# Autodesk Inventor assembly: obudowa_elektroniki_proper
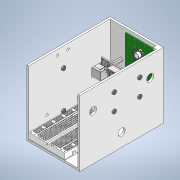
[picture p0: Inventor's stored thumbnail of the model, 180x180]
Saved by Autodesk Inventor 2020 (Build 240168000, 168)
## iProperties
Created: 2020-08-10
Part Number: obudowa_elektroniki_proper
Document SubType Name: Assembly
Designer: Hesekiel
Mass: 257.361 g
Surface Area: 1839.5 cm^2
Volume: 234.13 cm^3
Density: 1.09922 g/cm^3
Author: Hesekiel
## Documents named in this file (12)
- C:\Users\Hesekiel\Desktop\Equatorial-Mount-MUM\Mechanika\Mechanizm elewacji i elektronika Filip\CAD\obudowa_elektroniki_proper.iam
- C:\Users\Hesekiel\Desktop\Equatorial-Mount-MUM\Mechanika\Mechanizm elewacji i elektronika Filip\CAD\Sterownik silnika - Dual TB9051FTG.ipt
- C:\Users\Hesekiel\Desktop\Equatorial-Mount-MUM\Mechanika\Mechanizm elewacji i elektronika Filip\CAD\Konwerter step-down - D24V150FX.ipt
- C:\Users\Hesekiel\Desktop\Equatorial-Mount-MUM\Mechanika\Mechanizm elewacji i elektronika Filip\CAD\obudowa.ipt
- C:\Users\Hesekiel\Desktop\Equatorial-Mount-MUM\Mechanika\Mechanizm elewacji i elektronika Filip\CAD\arduino-uno-r3-1.snapshot.3\arduino uno.iam
- C:\Users\Hesekiel\Desktop\Equatorial-Mount-MUM\Mechanika\Mechanizm elewacji i elektronika Filip\CAD\DIN 912 - M3 x 0.5 x 6 x 4.75.ipt
- C:\Users\Hesekiel\Desktop\Equatorial-Mount-MUM\Mechanika\Mechanizm elewacji i elektronika Filip\CAD\DIN 934 - M3 x 0.5.ipt
- C:\Users\Hesekiel\Desktop\Equatorial-Mount-MUM\Mechanika\Mechanizm elewacji i elektronika Filip\CAD\Standoff_M3_14mm.ipt
- C:\Users\Hesekiel\Desktop\Equatorial-Mount-MUM\Mechanika\Mechanizm elewacji i elektronika Filip\CAD\HalfBreadboard.ipt
- C:\Users\Hesekiel\Desktop\Equatorial-Mount-MUM\Mechanika\Mechanizm elewacji i elektronika Filip\CAD\Battery 18650.ipt
- C:\Users\Hesekiel\Desktop\Equatorial-Mount-MUM\Mechanika\Mechanizm elewacji i elektronika Filip\CAD\battery-holder-for-2x-18650-1.snapshot.2\18650 holder 2x.ipt
- C:\Users\Hesekiel\Desktop\Equatorial-Mount-MUM\Mechanika\Mechanizm elewacji i elektronika Filip\CAD\DIN 912 - M3 x 0.5 x 10 x 8.75.ipt
## Components (39 placed, 11 different names)
1. Sterownik silnika - Dual TB9051FTG:1 — Mate:91, Mate:92, Mate:93, Mate:94, Mate:95, Mate:96, Mate:97
2. Konwerter step-down - D24V150FX:1 — Mate:55, Mate:56, Mate:65, Mate:66, Mate:67, Mate:68, Mate:69, Mate:70, Mate:71, Mate:72, Mate:73
3. obudowa:1 — Mate:1, Mate:2, Mate:30, Mate:31, Mate:32, Mate:33, Mate:34, Mate:35, Mate:36, Mate:37, Mate:39, Mate:40, Mate:41, Mate:42, Mate:44, Mate:50, Mate:51, Mate:52, Mate:55, Mate:56, Mate:57, Mate:58, Mate:59, Mate:60, Mate:61, Mate:62, Mate:63, Mate:64, Mate:75, Mate:76, Mate:77, Mate:81, Mate:85, Mate:86, Mate:88, Mate:91, Mate:92, Mate:95, Mate:99, Mate:100, Flush:3, Mate:101
4. arduino uno:1 [sub-assembly] — Mate:1, Mate:2, Mate:22, Mate:23, Mate:24, Mate:25, Mate:26, Mate:27, Mate:28, Mate:29, Mate:38
5. DIN 912 - replaced by DIN EN ISO 4762 M3 x 6:1 — Mate:22, Mate:23
6. DIN 912 - replaced by DIN EN ISO 4762 M3 x 6:2 — Mate:24, Mate:25
7. DIN 912 - replaced by DIN EN ISO 4762 M3 x 6:3 — Mate:26, Mate:27
8. DIN 912 - replaced by DIN EN ISO 4762 M3 x 6:4 — Mate:28, Mate:29
9. DIN 934 - replaced by DIN EN 24032/28673/28674 M3:1 — Mate:40, Mate:45
10. DIN 934 - replaced by DIN EN 24032/28673/28674 M3:2 — Mate:39, Mate:46
11. DIN 934 - replaced by DIN EN 24032/28673/28674 M3:3 — Mate:41, Mate:44
12. DIN 934 - replaced by DIN EN 24032/28673/28674 M3:4 — Mate:42, Mate:43
13. Standoff_M3_14mm:1 — Mate:30, Mate:31, Mate:38, Mate:43
14. Standoff_M3_14mm:2 — Mate:32, Mate:33
15. Standoff_M3_14mm:3 — Mate:34, Mate:35, Mate:45
16. Standoff_M3_14mm:4 — Mate:36, Mate:37, Mate:46
17. HalfBreadboard:1 — Mate:100, Flush:3, Mate:101
18. Battery 18650:1 — Mate:54, Flush:2
19. Battery 18650:2 — Mate:53, Flush:2
20. 18650 holder 2x:1 — Mate:50, Mate:51, Mate:52, Mate:53, Mate:54, Mate:83, Mate:84, Mate:89
21. DIN 934 - replaced by DIN EN 24032/28673/28674 M3:5 — Mate:57, Mate:61
22. DIN 934 - replaced by DIN EN 24032/28673/28674 M3:6 — Mate:58, Mate:62
23. DIN 934 - replaced by DIN EN 24032/28673/28674 M3:7 — Mate:59, Mate:63, Mate:65
24. DIN 934 - replaced by DIN EN 24032/28673/28674 M3:8 — Mate:60, Mate:64
25. DIN 912 - replaced by DIN EN ISO 4762 M3 x 10:1 — Mate:68, Mate:69, Mate:82
26. DIN 912 - replaced by DIN EN ISO 4762 M3 x 10:2 — Mate:70, Mate:71, Mate:79
27. DIN 912 - replaced by DIN EN ISO 4762 M3 x 10:3 — Mate:72, Mate:73, Mate:78
28. DIN 912 - replaced by DIN EN ISO 4762 M3 x 10:4 — Mate:66, Mate:67, Mate:80
29. DIN 934 - replaced by DIN EN 24032/28673/28674 M3:10 — Mate:75, Mate:79
30. DIN 934 - replaced by DIN EN 24032/28673/28674 M3:11 — Mate:76, Mate:78
31. DIN 934 - replaced by DIN EN 24032/28673/28674 M3:12 — Mate:77, Mate:80
32. DIN 934 - replaced by DIN EN 24032/28673/28674 M3:13 — Mate:81, Mate:82
33. DIN 912 - replaced by DIN EN ISO 4762 M3 x 6:5 — Mate:83, Mate:84, Mate:87
34. DIN 912 - replaced by DIN EN ISO 4762 M3 x 6:6 — Mate:88, Mate:89, Mate:90
35. DIN 934 - replaced by DIN EN 24032/28673/28674 M3:14 — Mate:85, Mate:87
36. DIN 934 - replaced by DIN EN 24032/28673/28674 M3:15 — Mate:86, Mate:90
37. DIN 934 - replaced by DIN EN 24032/28673/28674 M3:16 — Mate:93, Mate:94
38. DIN 912 - replaced by DIN EN ISO 4762 M3 x 10:5 — Mate:96, Mate:97, Mate:98
39. DIN 934 - replaced by DIN EN 24032/28673/28674 M3:17 — Mate:98, Mate:99
## Relationships (80: Mate 78, Flush 2)
- Mate:1: obudowa:1 ↔ arduino uno:1
- Mate:2: obudowa:1 ↔ arduino uno:1
- Mate:22: arduino uno:1 ↔ DIN 912 - replaced by DIN EN ISO 4762 M3 x 6:1
- Mate:23: arduino uno:1 ↔ DIN 912 - replaced by DIN EN ISO 4762 M3 x 6:1
- Mate:24: arduino uno:1 ↔ DIN 912 - replaced by DIN EN ISO 4762 M3 x 6:2
- Mate:25: arduino uno:1 ↔ DIN 912 - replaced by DIN EN ISO 4762 M3 x 6:2
- Mate:26: arduino uno:1 ↔ DIN 912 - replaced by DIN EN ISO 4762 M3 x 6:3
- Mate:27: arduino uno:1 ↔ DIN 912 - replaced by DIN EN ISO 4762 M3 x 6:3
- Mate:28: arduino uno:1 ↔ DIN 912 - replaced by DIN EN ISO 4762 M3 x 6:4
- Mate:29: arduino uno:1 ↔ DIN 912 - replaced by DIN EN ISO 4762 M3 x 6:4
- Mate:30: obudowa:1 ↔ Standoff_M3_14mm:1
- Mate:31: obudowa:1 ↔ Standoff_M3_14mm:1
- Mate:32: obudowa:1 ↔ Standoff_M3_14mm:2
- Mate:33: obudowa:1 ↔ Standoff_M3_14mm:2
- Mate:34: obudowa:1 ↔ Standoff_M3_14mm:3
- Mate:35: obudowa:1 ↔ Standoff_M3_14mm:3
- Mate:36: obudowa:1 ↔ Standoff_M3_14mm:4
- Mate:37: obudowa:1 ↔ Standoff_M3_14mm:4
- Mate:38: arduino uno:1 ↔ Standoff_M3_14mm:1
- Mate:39: obudowa:1 ↔ DIN 934 - replaced by DIN EN 24032/28673/28674 M3:2
- Mate:40: obudowa:1 ↔ DIN 934 - replaced by DIN EN 24032/28673/28674 M3:1
- Mate:41: obudowa:1 ↔ DIN 934 - replaced by DIN EN 24032/28673/28674 M3:3
- Mate:42: obudowa:1 ↔ DIN 934 - replaced by DIN EN 24032/28673/28674 M3:4
- Mate:43: DIN 934 - replaced by DIN EN 24032/28673/28674 M3:4 ↔ Standoff_M3_14mm:1
- Mate:44: obudowa:1 ↔ DIN 934 - replaced by DIN EN 24032/28673/28674 M3:3
- Mate:45: DIN 934 - replaced by DIN EN 24032/28673/28674 M3:1 ↔ Standoff_M3_14mm:3
- Mate:46: DIN 934 - replaced by DIN EN 24032/28673/28674 M3:2 ↔ Standoff_M3_14mm:4
- Mate:50: obudowa:1 ↔ 18650 holder 2x:1
- Mate:51: obudowa:1 ↔ 18650 holder 2x:1
- Mate:52: obudowa:1 ↔ 18650 holder 2x:1
- Mate:53: Battery 18650:2 ↔ 18650 holder 2x:1
- Mate:54: Battery 18650:1 ↔ 18650 holder 2x:1
- Flush:2: Battery 18650:1 ↔ Battery 18650:2
- Mate:55: Konwerter step-down - D24V150FX:1 ↔ obudowa:1
- Mate:56: Konwerter step-down - D24V150FX:1 ↔ obudowa:1
- Mate:57: obudowa:1 ↔ DIN 934 - replaced by DIN EN 24032/28673/28674 M3:5
- Mate:58: obudowa:1 ↔ DIN 934 - replaced by DIN EN 24032/28673/28674 M3:6
- Mate:59: obudowa:1 ↔ DIN 934 - replaced by DIN EN 24032/28673/28674 M3:7
- Mate:60: obudowa:1 ↔ DIN 934 - replaced by DIN EN 24032/28673/28674 M3:8
- Mate:61: obudowa:1 ↔ DIN 934 - replaced by DIN EN 24032/28673/28674 M3:5
- Mate:62: obudowa:1 ↔ DIN 934 - replaced by DIN EN 24032/28673/28674 M3:6
- Mate:63: obudowa:1 ↔ DIN 934 - replaced by DIN EN 24032/28673/28674 M3:7
- Mate:64: obudowa:1 ↔ DIN 934 - replaced by DIN EN 24032/28673/28674 M3:8
- Mate:65: Konwerter step-down - D24V150FX:1 ↔ DIN 934 - replaced by DIN EN 24032/28673/28674 M3:7
- Mate:66: Konwerter step-down - D24V150FX:1 ↔ DIN 912 - replaced by DIN EN ISO 4762 M3 x 10:4
- Mate:67: Konwerter step-down - D24V150FX:1 ↔ DIN 912 - replaced by DIN EN ISO 4762 M3 x 10:4
- Mate:68: Konwerter step-down - D24V150FX:1 ↔ DIN 912 - replaced by DIN EN ISO 4762 M3 x 10:1
- Mate:69: Konwerter step-down - D24V150FX:1 ↔ DIN 912 - replaced by DIN EN ISO 4762 M3 x 10:1
- Mate:70: Konwerter step-down - D24V150FX:1 ↔ DIN 912 - replaced by DIN EN ISO 4762 M3 x 10:2
- Mate:71: Konwerter step-down - D24V150FX:1 ↔ DIN 912 - replaced by DIN EN ISO 4762 M3 x 10:2
- Mate:72: Konwerter step-down - D24V150FX:1 ↔ DIN 912 - replaced by DIN EN ISO 4762 M3 x 10:3
- Mate:73: Konwerter step-down - D24V150FX:1 ↔ DIN 912 - replaced by DIN EN ISO 4762 M3 x 10:3
- Mate:75: obudowa:1 ↔ DIN 934 - replaced by DIN EN 24032/28673/28674 M3:10
- Mate:76: obudowa:1 ↔ DIN 934 - replaced by DIN EN 24032/28673/28674 M3:11
- Mate:77: obudowa:1 ↔ DIN 934 - replaced by DIN EN 24032/28673/28674 M3:12
- Mate:78: DIN 912 - replaced by DIN EN ISO 4762 M3 x 10:3 ↔ DIN 934 - replaced by DIN EN 24032/28673/28674 M3:11
- Mate:79: DIN 912 - replaced by DIN EN ISO 4762 M3 x 10:2 ↔ DIN 934 - replaced by DIN EN 24032/28673/28674 M3:10
- Mate:80: DIN 912 - replaced by DIN EN ISO 4762 M3 x 10:4 ↔ DIN 934 - replaced by DIN EN 24032/28673/28674 M3:12
- Mate:81: obudowa:1 ↔ DIN 934 - replaced by DIN EN 24032/28673/28674 M3:13
- Mate:82: DIN 912 - replaced by DIN EN ISO 4762 M3 x 10:1 ↔ DIN 934 - replaced by DIN EN 24032/28673/28674 M3:13
- Mate:83: 18650 holder 2x:1 ↔ DIN 912 - replaced by DIN EN ISO 4762 M3 x 6:5
- Mate:84: 18650 holder 2x:1 ↔ DIN 912 - replaced by DIN EN ISO 4762 M3 x 6:5
- Mate:85: obudowa:1 ↔ DIN 934 - replaced by DIN EN 24032/28673/28674 M3:14
- Mate:86: obudowa:1 ↔ DIN 934 - replaced by DIN EN 24032/28673/28674 M3:15
- Mate:87: DIN 912 - replaced by DIN EN ISO 4762 M3 x 6:5 ↔ DIN 934 - replaced by DIN EN 24032/28673/28674 M3:14
- Mate:88: obudowa:1 ↔ DIN 912 - replaced by DIN EN ISO 4762 M3 x 6:6
- Mate:89: 18650 holder 2x:1 ↔ DIN 912 - replaced by DIN EN ISO 4762 M3 x 6:6
- Mate:90: DIN 912 - replaced by DIN EN ISO 4762 M3 x 6:6 ↔ DIN 934 - replaced by DIN EN 24032/28673/28674 M3:15
- Mate:91: Sterownik silnika - Dual TB9051FTG:1 ↔ obudowa:1
- Mate:92: Sterownik silnika - Dual TB9051FTG:1 ↔ obudowa:1
- Mate:93: Sterownik silnika - Dual TB9051FTG:1 ↔ DIN 934 - replaced by DIN EN 24032/28673/28674 M3:16
- Mate:94: Sterownik silnika - Dual TB9051FTG:1 ↔ DIN 934 - replaced by DIN EN 24032/28673/28674 M3:16
- Mate:95: Sterownik silnika - Dual TB9051FTG:1 ↔ obudowa:1
- Mate:96: Sterownik silnika - Dual TB9051FTG:1 ↔ DIN 912 - replaced by DIN EN ISO 4762 M3 x 10:5
- Mate:97: Sterownik silnika - Dual TB9051FTG:1 ↔ DIN 912 - replaced by DIN EN ISO 4762 M3 x 10:5
- Mate:98: DIN 912 - replaced by DIN EN ISO 4762 M3 x 10:5 ↔ DIN 934 - replaced by DIN EN 24032/28673/28674 M3:17
- Mate:99: obudowa:1 ↔ DIN 934 - replaced by DIN EN 24032/28673/28674 M3:17
- Mate:100: obudowa:1 ↔ HalfBreadboard:1
- Flush:3: obudowa:1 ↔ HalfBreadboard:1
- Mate:101: obudowa:1 ↔ HalfBreadboard:1
